# Autodesk Inventor assembly: forearm
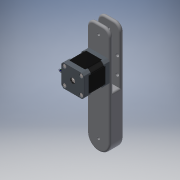
[picture p0: Inventor's stored thumbnail of the model, 180x180]
Saved by Autodesk Inventor 2019 (Build 230136000, 136)
## iProperties
Created: 2019-02-20
Part Number: forearm
Document SubType Name: Assembly
Designer: s-4036947
Author: s-4036947
## Documents named in this file (3)
- \\shares\studenthome\S-4036947\Inventor Files\fbd-arm\cad\arm.iam
- H:\Inventor Files\fbd-arm\cad\lower-arm.ipt
- \\shares\studenthome\S-4036947\Inventor Files\fbd-arm\cad\Nema17.ipt
## Components (2 placed, 2 different names)
1. lower-arm:1 — Mate:1, Mate:2, Mate:3
2. Nema17:1 — Mate:1, Mate:2, Mate:3
## Relationships (3: Mate 3)
- Mate:1: lower-arm:1 ↔ Nema17:1
- Mate:2: lower-arm:1 ↔ Nema17:1
- Mate:3: lower-arm:1 ↔ Nema17:1
